# Autodesk Inventor assembly: hegnspæl
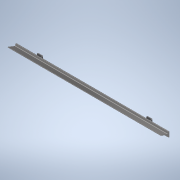
[picture p0: Inventor's stored thumbnail of the model, 180x180]
Saved by Autodesk Inventor 2020.1 (Build 241239000, 239)
## iProperties
Created: 2019-09-30
Part Number: hegnspæl
Document SubType Name: Assembly
Designer: Kristoffer Ek
Mass: 1821.47 g
Surface Area: 1100.09 cm^2
Volume: 232.034 cm^3
Density: 7.85 g/cm^3
_SolveAssemblyDoc: Frame Generator Solve Assembly
_Version: 15.0.0
Author: gust3763
## Documents named in this file (8)
- Y:\trappe\hegn\hegnspæl.iam
- hegnspæl.iam
- Y:\trappe\hegn\t-profil.ipt
- Y:\trappe\hegn\t-profil\Frame\Frame0002.iam
- Y:\trappe\hegn\hage.ipt
- Y:\trappe\hegn\gevindmuffe.ipt
- C:\Users\stoffer\Documents\Inventor\Content Center Files\R2020\en-US\ISO 4762(2)\ISO 4762 - M6 x 16ISO.ipt
- Y:\trappe\trappe.xlsx
## Components (6 placed, 5 different names)
1. t-profil:1
2. Frame0002:1 [sub-assembly] — Mate:1, Mate:2, Flush:1, Flush:2, Mate:3, Angle:1, Mate:4, Angle:2, Flush:5, Mate:5, Mate:6, Insert:1, Mate:8
3. hage:1 — Mate:1, Flush:2, Flush:6
4. hage:2 — Mate:2, Flush:1, Mate:5, Flush:6
5. gevindmuffe:1 — Mate:6, Insert:1, Mate:7
6. ISO 4762 M6 x 16:1 — Mate:7, Mate:8
## Relationships (15: Mate 8, Flush 4, Angle 2, Insert 1)
- Mate:1: Frame0002:1 ↔ hage:1
- Mate:2: Frame0002:1 ↔ hage:2
- Flush:1 (2.5 mm): Frame0002:1 ↔ hage:2
- Flush:2 (2.5 mm): Frame0002:1 ↔ hage:1
- Mate:3: Frame0002:1
- Angle:1 (0 deg): Frame0002:1
- Mate:4: Frame0002:1
- Angle:2 (0 deg): Frame0002:1
- Flush:5: Frame0002:1
- Mate:5 (-114 mm): Frame0002:1 ↔ hage:2
- Flush:6 (-630 mm): hage:1 ↔ hage:2
- Mate:6: Frame0002:1 ↔ gevindmuffe:1
- Insert:1: Frame0002:1 ↔ gevindmuffe:1
- Mate:7: gevindmuffe:1 ↔ ISO 4762 M6 x 16:1
- Mate:8: Frame0002:1 ↔ ISO 4762 M6 x 16:1
## Named parameters: trappevinkel = 34.3 deg, trappestifter_dia = 25 mm, trappestifter_huldia = 25.8 mm, trappestifter_skraa_huldia = 26.6 mm, trappestifter_laengde = 228 mm, perforeringsbredde = 6 mm, perforeringshulprocent = 80 mm, perforeringshullaengde = 62.8 mm, perforeringshullaengde_top = 61 mm, perforeringshullaengde_bund = 61.6 mm, perforeringsoffset = 8 mm, perforeringsoffset_top = 8 mm, perforeringsoffset_bund = 8 mm, laskehul_dia = 13 mm, haandfang_offset_fra_top = 90 mm, balusterhul_udvidelse = 1 mm, pladetykkelse = 3 mm, trinhoejde = 100 mm, trinbredde = 1884 mm
